# Autodesk Inventor assembly: zlozenie
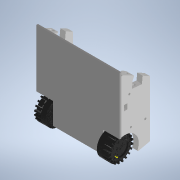
[picture p0: Inventor's stored thumbnail of the model, 180x180]
Saved by Autodesk Inventor 2022.3 (Build 263350000, 350)
## iProperties
Created: 2022-10-11
Part Number: zlozenie
Document SubType Name: Assembly
Designer: komputer
Author: komputer
## Documents named in this file (12)
- H:\ILYT_MS\zlozenie.iam
- H:\ILYT_MS\minisumopodsr.ipt
- H:\ILYT_MS\sciana_prawa_v4.ipt
- H:\ILYT_MS\n20 motor.ipt
- H:\ILYT_MS\koło_minisumo.ipt
- H:\ILYT_MS\pokrywa.ipt
- H:\ILYT_MS\pokrywa lewa.ipt
- H:\ILYT_MS\pokrywa prawa.ipt
- H:\ILYT_MS\uchwyt_nowy.ipt
- C:\Users\komputer\Downloads\Sharp_IR-Sensor.ipt
- H:\ILYT_MS\sciana_lewa_v5.ipt
- H:\ILYT_MS\pług_v2.ipt
## Components (14 placed, 11 different names)
1. minisumopodsr:1 — Flush:4, Mate:5, Mate:6, Flush:10, Flush:13, Mate:20, Mate:22, Flush:15, Mate:24, Mate:28, Mate:29, Flush:18, Flush:19
2. sciana_prawa_v4:1 — Flush:4, Mate:5, Mate:6, Flush:14, Mate:25, Flush:17, Mate:35
3. n20 motor:1 — Flush:10, Mate:17, Mate:18, Flush:16
4. n20 motor:2 — Mate:15, Mate:16
5. koło_minisumo:1 — Mate:17, Mate:18
6. koło_minisumo:2 — Mate:15, Mate:16
7. pokrywa:1 — Flush:13, Mate:20
8. pokrywa lewa:1 — Mate:22
9. pokrywa prawa:1 — Flush:14
10. uchwyt_nowy:1 — Flush:15, Mate:24, Flush:16
11. Sharp_IR-Sensor:1 — Mate:25, Mate:35
12. sciana_lewa_v5:1 — Flush:17, Mate:28, Mate:29, Mate:30, Mate:31, Mate:36
13. Sharp_IR-Sensor:2 — Mate:30, Mate:31, Mate:36
14. pług_v2:1 — Flush:18, Flush:19
## Relationships (25: Mate 16, Flush 9)
- Flush:4 (0.6 mm): minisumopodsr:1 ↔ sciana_prawa_v4:1
- Mate:5: minisumopodsr:1 ↔ sciana_prawa_v4:1
- Mate:6: minisumopodsr:1 ↔ sciana_prawa_v4:1
- Flush:10: minisumopodsr:1 ↔ n20 motor:1
- Mate:15: n20 motor:2 ↔ koło_minisumo:2
- Mate:16: n20 motor:2 ↔ koło_minisumo:2
- Mate:17: n20 motor:1 ↔ koło_minisumo:1
- Mate:18: n20 motor:1 ↔ koło_minisumo:1
- Flush:13: minisumopodsr:1 ↔ pokrywa:1
- Mate:20: minisumopodsr:1 ↔ pokrywa:1
- Mate:22: minisumopodsr:1 ↔ pokrywa lewa:1
- Flush:14: sciana_prawa_v4:1 ↔ pokrywa prawa:1
- Flush:15: minisumopodsr:1 ↔ uchwyt_nowy:1
- Mate:24: minisumopodsr:1 ↔ uchwyt_nowy:1
- Flush:16: n20 motor:1 ↔ uchwyt_nowy:1
- Mate:25: sciana_prawa_v4:1 ↔ Sharp_IR-Sensor:1
- Flush:17: sciana_prawa_v4:1 ↔ sciana_lewa_v5:1
- Mate:28: minisumopodsr:1 ↔ sciana_lewa_v5:1
- Mate:29 (0.6 mm): minisumopodsr:1 ↔ sciana_lewa_v5:1
- Mate:30: sciana_lewa_v5:1 ↔ Sharp_IR-Sensor:2
- Mate:31: sciana_lewa_v5:1 ↔ Sharp_IR-Sensor:2
- Mate:35: sciana_prawa_v4:1 ↔ Sharp_IR-Sensor:1
- Mate:36: sciana_lewa_v5:1 ↔ Sharp_IR-Sensor:2
- Flush:18: minisumopodsr:1 ↔ pług_v2:1
- Flush:19: minisumopodsr:1 ↔ pług_v2:1
